# Autodesk Inventor assembly: Leg_left
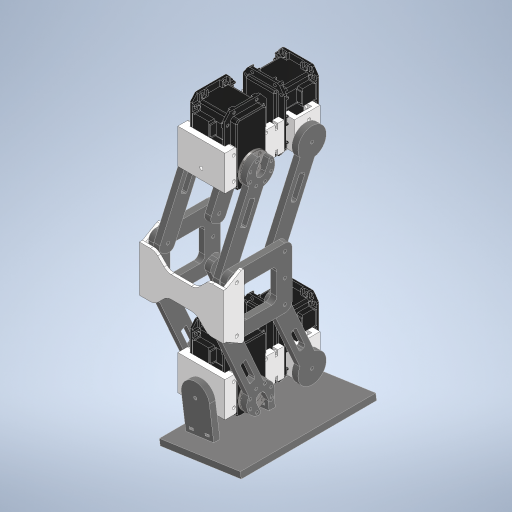
[picture p0: Inventor's stored thumbnail of the model, 512x512]
Saved by Autodesk Inventor 2024.3 (Build 283343000, 343)
## iProperties
Created: 2024-09-18
Part Number: Leg_left
Document SubType Name: Assembly
Designer: 구지현
Author: 구지현
## Documents named in this file (18)
- C:\Users\구지현\Desktop\19th_intern_kdy_robot\부품\Lower_Body\Leg\Leg_left.iam
- C:\Users\구지현\Desktop\19th_intern_kdy_robot\부품\Lower_Body\Leg\Back_Ankle.ipt
- C:\Users\구지현\Desktop\19th_intern_kdy_robot\부품\Lower_Body\Leg\Front_Ankle.ipt
- C:\Users\구지현\Desktop\19th_intern_kdy_robot\부품\Lower_Body\Leg\Knee.ipt
- C:\Users\구지현\Desktop\19th_intern_kdy_robot\부품\Lower_Body\Leg\Knee_Covers.ipt
- C:\Users\구지현\Desktop\19th_intern_kdy_robot\부품\Lower_Body\Leg\Leg_Connection_Parts_Back.ipt
- C:\Users\구지현\Desktop\19th_intern_kdy_robot\부품\Lower_Body\Leg\Leg_Connection_Parts_Front.ipt
- C:\Users\구지현\Desktop\19th_intern_kdy_robot\부품\Lower_Body\Leg\Leg_Foot_Connection_Parts.ipt
- C:\Users\구지현\Desktop\19th_intern_kdy_robot\부품\Lower_Body\Leg\Link_Fixation_Connector.ipt
- C:\Users\구지현\Desktop\19th_intern_kdy_robot\부품\Lower_Body\Leg\Vertical_Fixation_Set.iam
- C:\Users\구지현\Documents\카카오톡 받은 파일\Hardware\ROBOTIS(Inventor 2024 ver.)\다이나믹셀\MX-64T+idle.ipt.iam
- C:\Users\구지현\Documents\카카오톡 받은 파일\Hardware\ROBOTIS(Inventor 2024 ver.)\다이나믹셀\MX-106T+idle.ipt.iam
- C:\Users\구지현\Documents\카카오톡 받은 파일\Hardware\ROBOTIS(Inventor 2024 ver.)\혼\64-106Horn.ipt
- C:\Users\구지현\Desktop\19th_intern_kdy_robot\부품\Lower_Body\Leg\Link_Fixation_Connector_MIR.ipt
- Link_Fixation_Connector_left_left.ipt
- C:\Users\구지현\Desktop\19th_intern_kdy_robot\부품\Lower_Body\Leg\Foot_MIR.ipt
- MX-64T+idle.ipt
- MX-106T+idle.ipt
## Components (30 placed, 14 different names)
1. Back_Ankle:1 — 삽입:14, 플러쉬:14, 각도:9, 삽입:37
2. Knee:1 — 삽입:18, 삽입:19, 플러쉬:4, 플러쉬:5, 삽입:23, 삽입:28, 삽입:29, 삽입:33
3. Knee_Covers:1 — 삽입:28, 삽입:29, 삽입:30, 삽입:31
4. Leg_Connection_Parts_Back:1 — 각도:5, 플러쉬:1, 각도:6, 메이트:18, 플러쉬:3, 삽입:18
5. Leg_Connection_Parts_Front:1 — 메이트:6, 메이트:7, 각도:3, 각도:4, 각도:7, 플러쉬:2, 삽입:21
6. Leg_Foot_Connection_Parts:1 — 메이트:1, 메이트:2, 메이트:3, 메이트:4, 메이트:5, 삽입:35, 플러쉬:15
7. Link_Fixation_Connector:1 — 메이트:14, 메이트:15, 메이트:16, 메이트:17, 메이트:18
8. Vertical_Fixation_Set:1 [sub-assembly] — 삽입:5, 삽입:6, 삽입:7, 삽입:8, 삽입:9, 삽입:10, 삽입:11, 삽입:12
9. MX-64T+idle.ipt:1 [sub-assembly] — 삽입:4, 플러쉬:8, 삽입:24, 삽입:25, 삽입:26, 삽입:27, 플러쉬:10, 메이트:25, 메이트:26, 메이트:27, 메이트:28, 메이트:30, 메이트:31, 메이트:32, 메이트:33
10. MX-64T+idle.ipt:2 [sub-assembly] — 삽입:7, 삽입:8, 삽입:9, 삽입:10, 메이트:10, 메이트:11, 메이트:12, 메이트:13, 메이트:14, 메이트:15, 메이트:16, 메이트:17, 플러쉬:8, 플러쉬:10, 삽입:34
11. MX-106T+idle.ipt:1 [sub-assembly] — 삽입:2, 삽입:5, 삽입:6, 삽입:11, 삽입:12, 메이트:1, 메이트:2, 메이트:3, 메이트:4, 메이트:5, 메이트:8, 메이트:9, 플러쉬:7, 플러쉬:9
12. MX-106T+idle.ipt:2 [sub-assembly] — 삽입:1, 플러쉬:7, 메이트:22, 메이트:23, 메이트:24, 플러쉬:9, 메이트:35, 메이트:36
13. 64-106Horn:1 — 삽입:2, 메이트:6, 메이트:7
14. 64-106Horn:2 — 삽입:1, 메이트:20, 메이트:21
15. 64-106Horn:3 — 삽입:14, 삽입:34
16. 64-106Horn:4 — 삽입:4
17. Leg_Connection_Parts_Front:2 — 메이트:8, 메이트:9, 각도:3, 각도:4, 각도:6, 플러쉬:3, 삽입:19
18. Link_Fixation_Connector_left_left:1 — 메이트:10, 메이트:11, 메이트:12, 메이트:13, 메이트:19
19. Leg_Connection_Parts_Back:2 — 각도:5, 플러쉬:1, 각도:7, 메이트:19, 플러쉬:2, 삽입:20
20. Knee:2 — 삽입:20, 삽입:21, 플러쉬:4, 플러쉬:5, 삽입:22, 삽입:30, 삽입:31, 삽입:32
21. Leg_Connection_Parts_Front:3 — 삽입:22, 플러쉬:6, 메이트:20, 메이트:21, 플러쉬:11, 각도:8
22. Leg_Connection_Parts_Front:4 — 삽입:23, 플러쉬:6, 플러쉬:13
23. Vertical_Fixation_Set:2 [sub-assembly] — 메이트:22, 메이트:23, 메이트:24, 삽입:24, 삽입:25, 삽입:26, 삽입:27
24. Leg_Connection_Parts_Back:3 — 플러쉬:11, 각도:8, 삽입:32, 메이트:29, 플러쉬:12
25. Link_Fixation_Connector_left_left:2 — 메이트:25, 메이트:26, 메이트:27, 메이트:28, 메이트:29
26. Link_Fixation_Connector:2 — 메이트:30, 메이트:31, 메이트:32, 메이트:33, 메이트:34
27. Leg_Connection_Parts_Back:4 — 삽입:33, 플러쉬:12, 플러쉬:13, 메이트:34
28. Front_Ankle:2 — 삽입:35, 플러쉬:14, 각도:9, 삽입:36
29. Foot_left:1 — 삽입:36, 삽입:37
30. Leg_Foot_Connection_Parts:2 — 플러쉬:15, 메이트:35, 메이트:36
## Relationships (90: Mate 36, Insert 32, Flush 15, Angle 7)
- 삽입:1 [Insert]: MX-106T+idle.ipt:2 ↔ 64-106Horn:2
- 삽입:2 [Insert]: MX-106T+idle.ipt:1 ↔ 64-106Horn:1
- 삽입:4 [Insert]: MX-64T+idle.ipt:1 ↔ 64-106Horn:4
- 삽입:5 [Insert] (0.1 mm): Vertical_Fixation_Set:1 ↔ MX-106T+idle.ipt:1
- 삽입:6 [Insert] (0.1 mm): Vertical_Fixation_Set:1 ↔ MX-106T+idle.ipt:1
- 삽입:7 [Insert]: Vertical_Fixation_Set:1 ↔ MX-64T+idle.ipt:2
- 삽입:8 [Insert]: Vertical_Fixation_Set:1 ↔ MX-64T+idle.ipt:2
- 삽입:9 [Insert]: Vertical_Fixation_Set:1 ↔ MX-64T+idle.ipt:2
- 삽입:10 [Insert]: Vertical_Fixation_Set:1 ↔ MX-64T+idle.ipt:2
- 삽입:11 [Insert] (0.1 mm): Vertical_Fixation_Set:1 ↔ MX-106T+idle.ipt:1
- 삽입:12 [Insert] (0.1 mm): Vertical_Fixation_Set:1 ↔ MX-106T+idle.ipt:1
- 삽입:14 [Insert]: Back_Ankle:1 ↔ 64-106Horn:3
- 메이트:1 [Mate] (0.1 mm): Leg_Foot_Connection_Parts:1 ↔ MX-106T+idle.ipt:1
- 메이트:2 [Mate] (0.1 mm): Leg_Foot_Connection_Parts:1 ↔ MX-106T+idle.ipt:1
- 메이트:3 [Mate] (0.1 mm): Leg_Foot_Connection_Parts:1 ↔ MX-106T+idle.ipt:1
- 메이트:4 [Mate]: Leg_Foot_Connection_Parts:1 ↔ MX-106T+idle.ipt:1
- 메이트:5 [Mate]: Leg_Foot_Connection_Parts:1 ↔ MX-106T+idle.ipt:1
- 메이트:6 [Mate]: Leg_Connection_Parts_Front:1 ↔ 64-106Horn:1
- 메이트:7 [Mate]: Leg_Connection_Parts_Front:1 ↔ 64-106Horn:1
- 메이트:8 [Mate]: MX-106T+idle.ipt:1 ↔ Leg_Connection_Parts_Front:2
- 메이트:9 [Mate]: MX-106T+idle.ipt:1 ↔ Leg_Connection_Parts_Front:2
- 각도:3 [Angle] (0 deg): Leg_Connection_Parts_Front:1 ↔ Leg_Connection_Parts_Front:2
- 각도:4 [Angle] (0 deg): Leg_Connection_Parts_Front:1 ↔ Leg_Connection_Parts_Front:2
- 메이트:10 [Mate] (0.1 mm): MX-64T+idle.ipt:2 ↔ Link_Fixation_Connector_left_left:1
- 메이트:11 [Mate] (0.1 mm): MX-64T+idle.ipt:2 ↔ Link_Fixation_Connector_left_left:1
- 메이트:12 [Mate]: MX-64T+idle.ipt:2 ↔ Link_Fixation_Connector_left_left:1
- 메이트:13 [Mate]: MX-64T+idle.ipt:2 ↔ Link_Fixation_Connector_left_left:1
- 메이트:14 [Mate] (0.1 mm): Link_Fixation_Connector:1 ↔ MX-64T+idle.ipt:2
- 메이트:15 [Mate] (0.1 mm): Link_Fixation_Connector:1 ↔ MX-64T+idle.ipt:2
- 메이트:16 [Mate]: Link_Fixation_Connector:1 ↔ MX-64T+idle.ipt:2
- 메이트:17 [Mate]: Link_Fixation_Connector:1 ↔ MX-64T+idle.ipt:2
- 각도:5 [Angle] (0 deg): Leg_Connection_Parts_Back:1 ↔ Leg_Connection_Parts_Back:2
- 플러쉬:1 [Flush]: Leg_Connection_Parts_Back:1 ↔ Leg_Connection_Parts_Back:2
- 각도:6 [Angle] (0 deg): Leg_Connection_Parts_Back:1 ↔ Leg_Connection_Parts_Front:2
- 각도:7 [Angle] (0 deg): Leg_Connection_Parts_Front:1 ↔ Leg_Connection_Parts_Back:2
- 메이트:18 [Mate]: Leg_Connection_Parts_Back:1 ↔ Link_Fixation_Connector:1
- 메이트:19 [Mate]: Link_Fixation_Connector_left_left:1 ↔ Leg_Connection_Parts_Back:2
- 플러쉬:2 [Flush]: Leg_Connection_Parts_Front:1 ↔ Leg_Connection_Parts_Back:2
- 플러쉬:3 [Flush]: Leg_Connection_Parts_Back:1 ↔ Leg_Connection_Parts_Front:2
- 삽입:18 [Insert]: Knee:1 ↔ Leg_Connection_Parts_Back:1
- 삽입:19 [Insert]: Knee:1 ↔ Leg_Connection_Parts_Front:2
- 삽입:20 [Insert]: Leg_Connection_Parts_Back:2 ↔ Knee:2
- 삽입:21 [Insert]: Leg_Connection_Parts_Front:1 ↔ Knee:2
- 플러쉬:4 [Flush]: Knee:1 ↔ Knee:2
- 플러쉬:5 [Flush]: Knee:1 ↔ Knee:2
- 삽입:22 [Insert]: Knee:2 ↔ Leg_Connection_Parts_Front:3
- 삽입:23 [Insert]: Knee:1 ↔ Leg_Connection_Parts_Front:4
- 플러쉬:6 [Flush]: Leg_Connection_Parts_Front:3 ↔ Leg_Connection_Parts_Front:4
- 메이트:20 [Mate]: 64-106Horn:2 ↔ Leg_Connection_Parts_Front:3
- 메이트:21 [Mate]: 64-106Horn:2 ↔ Leg_Connection_Parts_Front:3
- 플러쉬:7 [Flush]: MX-106T+idle.ipt:1 ↔ MX-106T+idle.ipt:2
- 메이트:22 [Mate]: MX-106T+idle.ipt:2 ↔ Vertical_Fixation_Set:2
- 메이트:23 [Mate] (0.1 mm): MX-106T+idle.ipt:2 ↔ Vertical_Fixation_Set:2
- 메이트:24 [Mate]: MX-106T+idle.ipt:2 ↔ Vertical_Fixation_Set:2
- 플러쉬:8 [Flush]: MX-64T+idle.ipt:1 ↔ MX-64T+idle.ipt:2
- 삽입:24 [Insert]: MX-64T+idle.ipt:1 ↔ Vertical_Fixation_Set:2
- 삽입:25 [Insert]: MX-64T+idle.ipt:1 ↔ Vertical_Fixation_Set:2
- 삽입:26 [Insert]: MX-64T+idle.ipt:1 ↔ Vertical_Fixation_Set:2
- 삽입:27 [Insert]: MX-64T+idle.ipt:1 ↔ Vertical_Fixation_Set:2
- 플러쉬:9 [Flush]: MX-106T+idle.ipt:1 ↔ MX-106T+idle.ipt:2
- 플러쉬:10 [Flush]: MX-64T+idle.ipt:1 ↔ MX-64T+idle.ipt:2
- 삽입:28 [Insert]: Knee:1 ↔ Knee_Covers:1
- 삽입:29 [Insert]: Knee:1 ↔ Knee_Covers:1
- 삽입:30 [Insert]: Knee_Covers:1 ↔ Knee:2
- 삽입:31 [Insert]: Knee_Covers:1 ↔ Knee:2
- 플러쉬:11 [Flush]: Leg_Connection_Parts_Front:3 ↔ Leg_Connection_Parts_Back:3
- 각도:8 [Angle] (0 deg): Leg_Connection_Parts_Front:3 ↔ Leg_Connection_Parts_Back:3
- 삽입:32 [Insert]: Knee:2 ↔ Leg_Connection_Parts_Back:3
- 메이트:25 [Mate] (0.1 mm): MX-64T+idle.ipt:1 ↔ Link_Fixation_Connector_left_left:2
- 메이트:26 [Mate] (0.1 mm): MX-64T+idle.ipt:1 ↔ Link_Fixation_Connector_left_left:2
- 메이트:27 [Mate]: MX-64T+idle.ipt:1 ↔ Link_Fixation_Connector_left_left:2
- 메이트:28 [Mate]: MX-64T+idle.ipt:1 ↔ Link_Fixation_Connector_left_left:2
- 메이트:29 [Mate]: Leg_Connection_Parts_Back:3 ↔ Link_Fixation_Connector_left_left:2
- 삽입:33 [Insert]: Knee:1 ↔ Leg_Connection_Parts_Back:4
- 플러쉬:12 [Flush]: Leg_Connection_Parts_Back:3 ↔ Leg_Connection_Parts_Back:4
- 플러쉬:13 [Flush]: Leg_Connection_Parts_Front:4 ↔ Leg_Connection_Parts_Back:4
- 메이트:30 [Mate] (0.1 mm): MX-64T+idle.ipt:1 ↔ Link_Fixation_Connector:2
- 메이트:31 [Mate] (0.1 mm): MX-64T+idle.ipt:1 ↔ Link_Fixation_Connector:2
- 메이트:32 [Mate]: MX-64T+idle.ipt:1 ↔ Link_Fixation_Connector:2
- 메이트:33 [Mate]: MX-64T+idle.ipt:1 ↔ Link_Fixation_Connector:2
- 메이트:34 [Mate]: Link_Fixation_Connector:2 ↔ Leg_Connection_Parts_Back:4
- 삽입:34 [Insert]: MX-64T+idle.ipt:2 ↔ 64-106Horn:3
- 삽입:35 [Insert]: Leg_Foot_Connection_Parts:1 ↔ Front_Ankle:2
- 플러쉬:14 [Flush]: Back_Ankle:1 ↔ Front_Ankle:2
- 각도:9 [Angle] (0 deg): Back_Ankle:1 ↔ Front_Ankle:2
- 삽입:36 [Insert]: Front_Ankle:2 ↔ Foot_left:1
- 삽입:37 [Insert]: Back_Ankle:1 ↔ Foot_left:1
- 플러쉬:15 [Flush]: Leg_Foot_Connection_Parts:1 ↔ Leg_Foot_Connection_Parts:2
- 메이트:35 [Mate]: MX-106T+idle.ipt:2 ↔ Leg_Foot_Connection_Parts:2
- 메이트:36 [Mate]: MX-106T+idle.ipt:2 ↔ Leg_Foot_Connection_Parts:2
